# Autodesk Inventor assembly: Assembly(A)
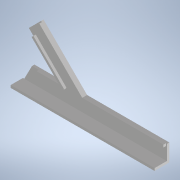
[picture p0: Inventor's stored thumbnail of the model, 180x180]
Saved by Autodesk Inventor 2020 (Build 240168000, 168)
## iProperties
Created: 2020-12-26
Part Number: Assembly(A)
Document SubType Name: Assembly
Designer: moham
Author: moham
## Documents named in this file (5)
- D:\Projects\MCT 131\The project\Track pieces\Section A\Assembly(A).iam
- D:\Projects\MCT 131\The project\Track pieces\Section A\A_Base.ipt
- D:\Projects\MCT 131\The project\Track pieces\Section A\A_LeftWall1(plan)_5.ipt
- D:\Projects\MCT 131\The project\Track pieces\Section A\A_LeftWall2(plan)_5.ipt
- D:\Projects\MCT 131\The project\Track pieces\Section A\A_RightWall.ipt
## Components (4 placed, 4 different names)
1. A_Base:1 — Mate:1, Flush:1, Flush:2, Mate:2, Flush:3, Mate:3, Flush:4
2. A_LeftWall1(plan)_5:1 — Mate:1, Flush:1, Flush:2
3. A_LeftWall2(plan)_5:1 — Mate:2
4. A_RightWall:1 — Flush:3, Mate:3, Flush:4
## Relationships (7: Flush 4, Mate 3)
- Mate:1: A_Base:1 ↔ A_LeftWall1(plan)_5:1
- Flush:1: A_Base:1 ↔ A_LeftWall1(plan)_5:1
- Flush:2: A_Base:1 ↔ A_LeftWall1(plan)_5:1
- Mate:2: A_Base:1 ↔ A_LeftWall2(plan)_5:1
- Flush:3: A_Base:1 ↔ A_RightWall:1
- Mate:3: A_Base:1 ↔ A_RightWall:1
- Flush:4: A_Base:1 ↔ A_RightWall:1
